# Autodesk Inventor assembly: Battery Cart Storage Assembly
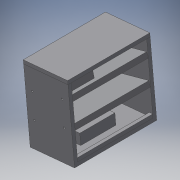
[picture p0: Inventor's stored thumbnail of the model, 180x180]
Saved by Autodesk Inventor 2018 (Build 220112000, 112)
## iProperties
Created: 2018-12-10
Part Number: Battery Cart Storage Assembly
Document SubType Name: Assembly
Designer: Gabriel
Author: Gabriel
## Documents named in this file (7)
- C:\Users\Gabriel\Documents\GitHub\2019CAD\Gab Battery Cart\Battery Cart Storage Assembly.iam
- C:\Users\Gabriel\Documents\GitHub\2019CAD\Gab Battery Cart\Cart Box.ipt
- C:\Users\Gabriel\Documents\GitHub\2019CAD\Gab Battery Cart\Cart Shelf.ipt
- C:\Users\Gabriel\Documents\GitHub\2019CAD\Gab Battery Cart\Bottom Bumper.ipt
- C:\Users\Gabriel\Downloads\BatteryModel.ipt
- C:\Users\Gabriel\Documents\GitHub\2019CAD\Top Of Cart.ipt
- C:\Users\Gabriel\Documents\GitHub\2019CAD\Battery Charger Repreentation.ipt
## Components (10 placed, 6 different names)
1. Cart Box:1 — Mate:1, Mate:2, Mate:3, Mate:4, Mate:5, Mate:6, Mate:7, Mate:8, Mate:12, Mate:13, Mate:14, Mate:15
2. Cart Shelf:1 — Mate:1, Mate:2, Mate:11
3. Cart Shelf:2 — Mate:5, Mate:6
4. Cart Shelf:3 — Mate:3, Mate:4
5. Bottom Bumper:1 — Mate:7, Mate:8
6. BatteryModel:1
7. BatteryModel:2 — Mate:11
8. BatteryModel:3
9. Top Of Cart:1 — Mate:12, Mate:13, Mate:14
10. Battery Charger Repreentation:1 — Mate:15
## Relationships (13: Mate 13)
- Mate:1: Cart Box:1 ↔ Cart Shelf:1
- Mate:2: Cart Box:1 ↔ Cart Shelf:1
- Mate:3: Cart Box:1 ↔ Cart Shelf:3
- Mate:4: Cart Box:1 ↔ Cart Shelf:3
- Mate:5: Cart Box:1 ↔ Cart Shelf:2
- Mate:6: Cart Box:1 ↔ Cart Shelf:2
- Mate:7: Cart Box:1 ↔ Bottom Bumper:1
- Mate:8: Cart Box:1 ↔ Bottom Bumper:1
- Mate:11: Cart Shelf:1 ↔ BatteryModel:2
- Mate:12: Cart Box:1 ↔ Top Of Cart:1
- Mate:13: Cart Box:1 ↔ Top Of Cart:1
- Mate:14 (0.2286 mm): Cart Box:1 ↔ Top Of Cart:1
- Mate:15: Cart Box:1 ↔ Battery Charger Repreentation:1
